# Autodesk Inventor assembly: Platform assembly with IR
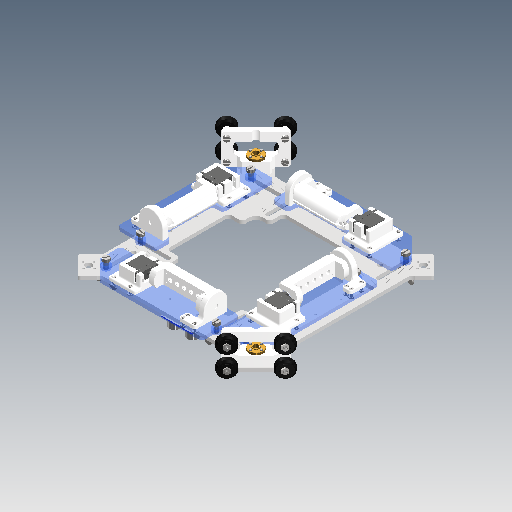
[picture p0: Inventor's stored thumbnail of the model, 512x512]
Saved by Autodesk Inventor 2020 (Build 240168000, 168)
## iProperties
Created: 2020-12-15
Part Number: Platform assembly with IR
Document SubType Name: Assembly
Designer: ferrerx
Author: ferrerx
## Documents named in this file (9)
- C:\Users\ferrerx\Desktop\Prieto-Godino Lab\Drosophila Larvae Behavioural Device\Device design V3\Inventor Assembly\Platform assembly with IR.iam
- C:\Users\ferrerx\Desktop\Prieto-Godino Lab\Drosophila Larvae Behavioural Device\Device design V3\Inventor Assembly\Light sources platform.ipt
- C:\Users\ferrerx\Desktop\Prieto-Godino Lab\Drosophila Larvae Behavioural Device\Device design V3\Inventor Assembly\Cart assembly.iam
- C:\Users\ferrerx\Documents\Inventor\Content Center Files\R2020\en-US\AS 1427(05)\AS 1427 - M3 x 25(5) II.ipt
- C:\Users\ferrerx\Desktop\Prieto-Godino Lab\Drosophila Larvae Behavioural Device\Device design V3\Inventor Assembly\IR linear array assembly.iam
- C:\Users\ferrerx\Documents\Inventor\Content Center Files\R2020\en-US\AS 1427(10)\AS 1427 - M6 x 25(7).ipt
- C:\Users\ferrerx\Documents\Inventor\Content Center Files\R2020\en-US\CNS 4373\CNS 4373 - M 6.ipt
- C:\Users\ferrerx\Desktop\Prieto-Godino Lab\Drosophila Larvae Behavioural Device\Device design V3\Inventor Assembly\Ultrasonic sensor holder.ipt
- C:\Users\ferrerx\Desktop\Prieto-Godino Lab\Drosophila Larvae Behavioural Device\Device design V3\Inventor Assembly\Ultrasonic sensor.ipt
## Components (33 placed, 8 different names)
1. Light sources platform:1 — Mate:1, Mate:2, Angle:1, Mate:3, Mate:4, Angle:2, Mate:6, Mate:7, Mate:8, Mate:9, Mate:10, Mate:11, Mate:12, Mate:13, Mate:14, Mate:15, Mate:16, Mate:17, Mate:18, Mate:19, Mate:20, Mate:21, Mate:22, Mate:25, Mate:26, Mate:27, Mate:28, Mate:29, Mate:30, Mate:31, Mate:32, Mate:57, Mate:58, Mate:59, Mate:60, Mate:61, Mate:62, Mate:63, Mate:64, Mate:65, Mate:66, Mate:67
2. Cart assembly:1 [sub-assembly] — Mate:1, Mate:2, Angle:1, Mate:5
3. Cart assembly:2 [sub-assembly] — Mate:3, Mate:4, Angle:2
4. AS 1427 H - Metric M3 x 25:1 — Mate:5, Mate:6
5. AS 1427 H - Metric M3 x 25:2 — Mate:7, Mate:19
6. AS 1427 H - Metric M3 x 25:3 — Mate:9, Mate:20
7. AS 1427 H - Metric M3 x 25:4 — Mate:8, Mate:18
8. AS 1427 H - Metric M3 x 25:5 — Mate:12, Mate:16
9. AS 1427 H - Metric M3 x 25:6 — Mate:10, Mate:17
10. AS 1427 H - Metric M3 x 25:7 — Mate:13, Mate:14
11. AS 1427 H - Metric M3 x 25:8 — Mate:11, Mate:15
12. IR linear array assembly:1 [sub-assembly] — Mate:25, Mate:26, Mate:29, Mate:37, Mate:38, Mate:47, Mate:48
13. IR linear array assembly:2 [sub-assembly] — Mate:27, Mate:28, Mate:30, Mate:39, Mate:40, Mate:45, Mate:46
14. IR linear array assembly:3 [sub-assembly] — Mate:31, Mate:41, Mate:42, Mate:43, Mate:44
15. IR linear array assembly:4 [sub-assembly] — Mate:21, Mate:22, Mate:32, Mate:33, Mate:34, Mate:35, Mate:36
16. AS 1427 (8) - Metric M6 x 25:1 — Mate:33, Mate:34, Mate:50
17. AS 1427 (8) - Metric M6 x 25:2 — Mate:35, Mate:36, Mate:52
18. AS 1427 (8) - Metric M6 x 25:3 — Mate:37, Mate:48, Mate:49
19. AS 1427 (8) - Metric M6 x 25:4 — Mate:42, Mate:43, Mate:53
20. AS 1427 (8) - Metric M6 x 25:5 — Mate:39, Mate:46, Mate:56
21. AS 1427 (8) - Metric M6 x 25:6 — Mate:41, Mate:44, Mate:54
22. AS 1427 (8) - Metric M6 x 25:7 — Mate:40, Mate:45, Mate:55
23. AS 1427 (8) - Metric M6 x 25:8 — Mate:38, Mate:47, Mate:51
24. CNS 4373 M 6:1 — Mate:49, Mate:57
25. CNS 4373 M 6:2 — Mate:50, Mate:58
26. CNS 4373 M 6:3 — Mate:52, Mate:60
27. CNS 4373 M 6:4 — Mate:51, Mate:62
28. CNS 4373 M 6:5 — Mate:56, Mate:63
29. CNS 4373 M 6:6 — Mate:55, Mate:64
30. CNS 4373 M 6:7 — Mate:53, Mate:59
31. CNS 4373 M 6:8 — Mate:54, Mate:61
32. Ultrasonic sensor holder:1 — Mate:65, Mate:66, Mate:67, Mate:68, Mate:69, Mate:70
33. Ultrasonic sensor:1 — Mate:68, Mate:69, Mate:70
## Relationships (70: Mate 68, Angle 2)
- Mate:1: Light sources platform:1 ↔ Cart assembly:1
- Mate:2: Light sources platform:1 ↔ Cart assembly:1
- Angle:1 (0 deg): Light sources platform:1 ↔ Cart assembly:1
- Mate:3: Light sources platform:1 ↔ Cart assembly:2
- Mate:4: Light sources platform:1 ↔ Cart assembly:2
- Angle:2 (0 deg): Light sources platform:1 ↔ Cart assembly:2
- Mate:5: Cart assembly:1 ↔ AS 1427 H - Metric M3 x 25:1
- Mate:6: Light sources platform:1 ↔ AS 1427 H - Metric M3 x 25:1
- Mate:7: Light sources platform:1 ↔ AS 1427 H - Metric M3 x 25:2
- Mate:8: Light sources platform:1 ↔ AS 1427 H - Metric M3 x 25:4
- Mate:9: Light sources platform:1 ↔ AS 1427 H - Metric M3 x 25:3
- Mate:10: Light sources platform:1 ↔ AS 1427 H - Metric M3 x 25:6
- Mate:11: Light sources platform:1 ↔ AS 1427 H - Metric M3 x 25:8
- Mate:12: Light sources platform:1 ↔ AS 1427 H - Metric M3 x 25:5
- Mate:13: Light sources platform:1 ↔ AS 1427 H - Metric M3 x 25:7
- Mate:14: Light sources platform:1 ↔ AS 1427 H - Metric M3 x 25:7
- Mate:15: Light sources platform:1 ↔ AS 1427 H - Metric M3 x 25:8
- Mate:16: Light sources platform:1 ↔ AS 1427 H - Metric M3 x 25:5
- Mate:17: Light sources platform:1 ↔ AS 1427 H - Metric M3 x 25:6
- Mate:18: Light sources platform:1 ↔ AS 1427 H - Metric M3 x 25:4
- Mate:19: Light sources platform:1 ↔ AS 1427 H - Metric M3 x 25:2
- Mate:20: Light sources platform:1 ↔ AS 1427 H - Metric M3 x 25:3
- Mate:21: Light sources platform:1 ↔ IR linear array assembly:4
- Mate:22: Light sources platform:1 ↔ IR linear array assembly:4
- Mate:25: Light sources platform:1 ↔ IR linear array assembly:1
- Mate:26: Light sources platform:1 ↔ IR linear array assembly:1
- Mate:27: Light sources platform:1 ↔ IR linear array assembly:2
- Mate:28: Light sources platform:1 ↔ IR linear array assembly:2
- Mate:29: Light sources platform:1 ↔ IR linear array assembly:1
- Mate:30: Light sources platform:1 ↔ IR linear array assembly:2
- Mate:31: Light sources platform:1 ↔ IR linear array assembly:3
- Mate:32: Light sources platform:1 ↔ IR linear array assembly:4
- Mate:33: IR linear array assembly:4 ↔ AS 1427 (8) - Metric M6 x 25:1
- Mate:34: IR linear array assembly:4 ↔ AS 1427 (8) - Metric M6 x 25:1
- Mate:35: IR linear array assembly:4 ↔ AS 1427 (8) - Metric M6 x 25:2
- Mate:36: IR linear array assembly:4 ↔ AS 1427 (8) - Metric M6 x 25:2
- Mate:37: IR linear array assembly:1 ↔ AS 1427 (8) - Metric M6 x 25:3
- Mate:38: IR linear array assembly:1 ↔ AS 1427 (8) - Metric M6 x 25:8
- Mate:39: IR linear array assembly:2 ↔ AS 1427 (8) - Metric M6 x 25:5
- Mate:40: IR linear array assembly:2 ↔ AS 1427 (8) - Metric M6 x 25:7
- Mate:41: IR linear array assembly:3 ↔ AS 1427 (8) - Metric M6 x 25:6
- Mate:42: IR linear array assembly:3 ↔ AS 1427 (8) - Metric M6 x 25:4
- Mate:43: IR linear array assembly:3 ↔ AS 1427 (8) - Metric M6 x 25:4
- Mate:44: IR linear array assembly:3 ↔ AS 1427 (8) - Metric M6 x 25:6
- Mate:45: IR linear array assembly:2 ↔ AS 1427 (8) - Metric M6 x 25:7
- Mate:46: IR linear array assembly:2 ↔ AS 1427 (8) - Metric M6 x 25:5
- Mate:47: IR linear array assembly:1 ↔ AS 1427 (8) - Metric M6 x 25:8
- Mate:48: IR linear array assembly:1 ↔ AS 1427 (8) - Metric M6 x 25:3
- Mate:49: AS 1427 (8) - Metric M6 x 25:3 ↔ CNS 4373 M 6:1
- Mate:50: AS 1427 (8) - Metric M6 x 25:1 ↔ CNS 4373 M 6:2
- Mate:51: AS 1427 (8) - Metric M6 x 25:8 ↔ CNS 4373 M 6:4
- Mate:52: AS 1427 (8) - Metric M6 x 25:2 ↔ CNS 4373 M 6:3
- Mate:53: AS 1427 (8) - Metric M6 x 25:4 ↔ CNS 4373 M 6:7
- Mate:54: AS 1427 (8) - Metric M6 x 25:6 ↔ CNS 4373 M 6:8
- Mate:55: AS 1427 (8) - Metric M6 x 25:7 ↔ CNS 4373 M 6:6
- Mate:56: AS 1427 (8) - Metric M6 x 25:5 ↔ CNS 4373 M 6:5
- Mate:57: Light sources platform:1 ↔ CNS 4373 M 6:1
- Mate:58: Light sources platform:1 ↔ CNS 4373 M 6:2
- Mate:59: Light sources platform:1 ↔ CNS 4373 M 6:7
- Mate:60: Light sources platform:1 ↔ CNS 4373 M 6:3
- Mate:61: Light sources platform:1 ↔ CNS 4373 M 6:8
- Mate:62: Light sources platform:1 ↔ CNS 4373 M 6:4
- Mate:63: Light sources platform:1 ↔ CNS 4373 M 6:5
- Mate:64: Light sources platform:1 ↔ CNS 4373 M 6:6
- Mate:65: Light sources platform:1 ↔ Ultrasonic sensor holder:1
- Mate:66: Light sources platform:1 ↔ Ultrasonic sensor holder:1
- Mate:67: Light sources platform:1 ↔ Ultrasonic sensor holder:1
- Mate:68: Ultrasonic sensor holder:1 ↔ Ultrasonic sensor:1
- Mate:69: Ultrasonic sensor holder:1 ↔ Ultrasonic sensor:1
- Mate:70: Ultrasonic sensor holder:1 ↔ Ultrasonic sensor:1
